# Autodesk Inventor assembly: ElectronicLoad
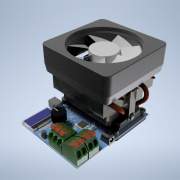
[picture p0: Inventor's stored thumbnail of the model, 180x180]
Saved by Autodesk Inventor 2021 (Build 250183000, 183)
## iProperties
Created: 2020-02-06
Part Number: ElectronicLoad
Document SubType Name: Assembly
Designer: Bradley
Author: Bradley
## Documents named in this file (42)
- C:\Users\Bradley\Documents\GitHub\Resources\Subsystems\Electronics\Testing\ElectronicLoad\CADModel\Native\ElectronicLoad.iam
- C:\Users\Bradley\Documents\GitHub\Resources\Subsystems\Electronics\Testing\ElectronicLoad\CADModel\Native\ElectronicLoad_PCB.ipt
- C:\Users\Bradley\Documents\GitHub\Resources\SupplierDocuments\05 - Connectors THT\05-0005\05-0005.ipt
- C:\Users\Bradley\Documents\GitHub\Resources\SupplierDocuments\05 - Connectors THT\05-0011\05-0011.ipt
- C:\Users\Bradley\Documents\GitHub\Resources\SupplierDocuments\05 - Connectors THT\05-0008\05-0008.ipt
- C:\Users\Bradley\Documents\GitHub\Resources\SupplierDocuments\05 - Connectors THT\05-0009\05-0009.ipt
- C:\Users\Bradley\Documents\GitHub\Resources\SupplierDocuments\04 - Connectors SMT\04-0004\04-0004.ipt
- C:\Users\Bradley\Documents\GitHub\Resources\SupplierDocuments\66 - Sensor\66-0006\66-0006.iam
- C:\Users\Bradley\Documents\GitHub\Resources\SupplierDocuments\03 - Board, Module, etc\03-0001\03-0001.ipt
- C:\Users\Bradley\Documents\GitHub\Resources\SupplierDocuments\05 - Connectors THT\05-0004\05-0004.ipt
- C:\Users\Bradley\Documents\GitHub\Resources\SupplierDocuments\61 - µController (and CLPD, FPGA,  etc.)\61-0002\61-0002.ipt
- C:\Users\Bradley\Documents\GitHub\Resources\SupplierDocuments\49 - Electromechanical\49-0005\49-0005.iam
- C:\Users\Bradley\Documents\GitHub\Resources\SupplierDocuments\48 - Hardware\48-0003\48-0003.iam
- C:\Users\Bradley\Documents\GitHub\Resources\SupplierDocuments\56 - Transistor FET\56-0008\56-0008-DOWN.ipt
- C:\Users\Bradley\Documents\GitHub\Resources\SupplierDocuments\23 - Resistor 3216\23-5m00\23-5m00.ipt
- C:\Users\Bradley\Documents\GitHub\Resources\SupplierDocuments\21 - Resistor 1608\21-0000\21-0000.ipt
- C:\Users\Bradley\Documents\GitHub\Resources\SupplierDocuments\36 - Ferrite\36-152A\36-152A.ipt
- C:\Users\Bradley\Documents\GitHub\Resources\SupplierDocuments\11 - Capacitor Ceramic 1608\11-105B\11-105B.ipt
- C:\Users\Bradley\Documents\GitHub\Resources\SupplierDocuments\21 - Resistor 1608\21-1001\21-1001.ipt
- C:\Users\Bradley\Documents\GitHub\Resources\SupplierDocuments\11 - Capacitor Ceramic 1608\11-102B\11-102B.ipt
- C:\Users\Bradley\Documents\GitHub\Resources\SupplierDocuments\16 - Capacitor Tantalum SMT\16-475A\16-475A.ipt
- C:\Users\Bradley\Documents\GitHub\Resources\SupplierDocuments\40 - Crystal SMT\40-805A\40-805A.ipt
- C:\Users\Bradley\Documents\GitHub\Resources\SupplierDocuments\21 - Resistor 1608\21-1002\21-1002.ipt
- C:\Users\Bradley\Documents\GitHub\Resources\SupplierDocuments\26 - Resistor Misc\26-0000\26-0000.ipt
- C:\Users\Bradley\Documents\GitHub\Resources\SupplierDocuments\11 - Capacitor Ceramic 1608\11-103A\11-103A.ipt
- C:\Users\Bradley\Documents\GitHub\Resources\SupplierDocuments\11 - Capacitor Ceramic 1608\11-100A\11-100A.ipt
- C:\Users\Bradley\Documents\GitHub\Resources\SupplierDocuments\21 - Resistor 1608\21-27.0\21-27.0.ipt
- C:\Users\Bradley\Documents\GitHub\Resources\SupplierDocuments\21 - Resistor 1608\21-3002\21-3002.ipt
- C:\Users\Bradley\Documents\GitHub\Resources\SupplierDocuments\21 - Resistor 1608\21-4702\21-4702.ipt
- C:\Users\Bradley\Documents\GitHub\Resources\SupplierDocuments\11 - Capacitor Ceramic 1608\11-470A\11-470A.ipt
- C:\Users\Bradley\Documents\GitHub\Resources\SupplierDocuments\21 - Resistor 1608\21-0.05\21-0.05.ipt
- C:\Users\Bradley\Documents\GitHub\Resources\SupplierDocuments\11 - Capacitor Ceramic 1608\11-104A\11-104A.ipt
- C:\Users\Bradley\Documents\GitHub\Resources\SupplierDocuments\21 - Resistor 1608\21-0.51\21-0.51.ipt
- C:\Users\Bradley\Documents\GitHub\Resources\SupplierDocuments\08 - Amplifier (excluding RF)\08-0002\08-0002.ipt
- C:\Users\Bradley\Documents\GitHub\Resources\SupplierDocuments\09 - Communication IC\09-0002\09-0002.ipt
- C:\Users\Bradley\Documents\GitHub\Resources\SupplierDocuments\63 - LED SMT\63-0001\63-0001.ipt
- C:\Users\Bradley\Documents\GitHub\Resources\SupplierDocuments\08 - Amplifier (excluding RF)\08-0003\08-0003.ipt
- C:\Users\Bradley\Documents\GitHub\Resources\SupplierDocuments\60 - Power IC\60-0009\60-0009.ipt
- C:\Users\Bradley\Documents\GitHub\Resources\SupplierDocuments\53 - Diode Misc\53-0001\53-0001.ipt
- C:\Users\Bradley\Documents\GitHub\Resources\SupplierDocuments\63 - LED SMT\63-0002\63-0002.ipt
- C:\Users\Bradley\Documents\GitHub\Resources\SupplierDocuments\56 - Transistor FET\56-0009\56-0009.ipt
- C:\Users\Bradley\Documents\GitHub\Resources\SupplierDocuments\60 - Power IC\60-0012\60-0012.ipt
## Components (90 placed, 41 different names)
1. ElectronicLoad_PCB:1 — Mate:6, Mate:7, Mate:8, Mate:9, Mate:10, Mate:11, Mate:12, Mate:13, Mate:14, Mate:15, Mate:16, Insert:1, Insert:2, Insert:3, Insert:4, Insert:5, Mate:27, Mate:34, Mate:35, Mate:36, Mate:37, Mate:38, Mate:39, Mate:50, Mate:53, Mate:55, Mate:56, Mate:57, Mate:58, Mate:59, Mate:60, Mate:61, Mate:62, Mate:63, Mate:64, Mate:75, Mate:76, Mate:77, Mate:78, Mate:79, Mate:80, Mate:81, Mate:95, Mate:96, Mate:99, Mate:100, Mate:105, Mate:106, Mate:108, Mate:109, Mate:110, Mate:111, Mate:120, Mate:121, Mate:125, Mate:127, Mate:128, Mate:133, Mate:134, Mate:139, Mate:140, Mate:141, Mate:148, Mate:150, Mate:151, Mate:156, Mate:158, Mate:159, Mate:160, Mate:161, Mate:162, Mate:163, Mate:164, Mate:165, Mate:166, Mate:167, Mate:168, Mate:169, Mate:186, Mate:189, Mate:191, Mate:194, Mate:195, Mate:200, Mate:201, Mate:204, Mate:207, Mate:208, Mate:209, Mate:212, Mate:213, Mate:215
2. 08-0002:1 — Mate:189, Mate:190, Flush:52
3. 09-0002:1 — Mate:191, Mate:192, Mate:193
4. 63-0001:1 — Mate:194, Mate:196, Mate:197
5. 63-0001:2 — Mate:195, Mate:198, Mate:199
6. 08-0003:1 — Mate:200, Mate:202, Mate:203
7. 08-0003:2 — Mate:201, Flush:53, Flush:54
8. 60-0009:1 — Mate:204, Mate:205, Mate:206
9. 53-0001:1 — Mate:207, Flush:55, Flush:56
10. 53-0001:2 — Mate:208, Flush:57, Flush:58
11. 63-0002:1 — Mate:209, Mate:210, Mate:211
12. 56-0009:1 — Mate:212, Mate:214, Flush:59
13. 56-0009:2 — Mate:213, Flush:60, Flush:61
14. 60-0012:1 — Mate:215, Flush:62, Flush:63
15. 21-0.51:1 — Mate:186, Mate:187, Mate:188
16. 11-104A:1 — Mate:158, Mate:170, Flush:44
17. 11-104A:2 — Mate:159, Mate:171, Mate:172
18. 11-104A:3 — Mate:160, Mate:173, Mate:174
19. 11-104A:4 — Mate:161, Mate:175, Mate:176
20. 11-104A:5 — Mate:162, Mate:177, Mate:178
21. 11-104A:6 — Mate:163, Mate:179, Flush:45
22. 11-104A:7 — Mate:164, Mate:180, Flush:46
23. 11-104A:8 — Mate:165, Mate:181, Flush:47
24. 11-104A:9 — Mate:166, Mate:182, Flush:48
25. 11-104A:10 — Mate:167, Mate:183, Flush:49
26. 11-104A:11 — Mate:168, Mate:184, Flush:50
27. 11-104A:12 — Mate:169, Mate:185, Flush:51
28. 21-0.05:1 — Mate:156, Mate:157, Flush:43
29. 11-470A:1 — Mate:150, Mate:152, Mate:153
30. 11-470A:2 — Mate:151, Mate:154, Mate:155
31. 21-4702:1 — Mate:148, Mate:149, Flush:42
32. 21-3002:1 — Mate:139, Mate:142, Mate:143
33. 21-3002:2 — Mate:140, Mate:144, Mate:145
34. 21-3002:3 — Mate:141, Mate:146, Mate:147
35. 21-27.0:1 — Mate:133, Mate:135, Mate:136
36. 21-27.0:2 — Mate:134, Mate:137, Mate:138
37. 11-100A:1 — Mate:127, Mate:129, Mate:130
38. 11-100A:2 — Mate:128, Mate:131, Mate:132
39. 11-103A:1 — Mate:125, Mate:126, Flush:41
40. 26-0000:1 — Mate:120, Mate:122, Flush:40
41. 26-0000:2 — Mate:121, Mate:123, Mate:124
42. 21-1002:1 — Mate:108, Mate:112, Mate:113
43. 21-1002:2 — Mate:109, Mate:114, Mate:115
44. 21-1002:3 — Mate:110, Mate:116, Mate:117
45. 21-1002:4 — Mate:111, Mate:118, Mate:119
46. 40-805A:1 — Mate:106, Mate:107, Flush:39
47. 23-5m00:2 — Mate:105, Flush:37, Flush:38
48. 16-475A:1 — Mate:99, Mate:101, Mate:102
49. 16-475A:2 — Mate:100, Mate:103, Mate:104
50. 11-102B:1 — Mate:95, Mate:97, Flush:35
51. 11-102B:2 — Mate:96, Mate:98, Flush:36
52. 21-1001:1 — Mate:75, Mate:82, Mate:83
53. 21-1001:2 — Mate:76, Mate:84, Mate:85
54. 21-1001:3 — Mate:77, Mate:86, Mate:87
55. 21-1001:4 — Mate:78, Mate:88, Mate:89
56. 21-1001:5 — Mate:79, Mate:90, Mate:91
57. 21-1001:6 — Mate:80, Mate:92, Mate:93
58. 21-1001:7 — Mate:81, Mate:94, Flush:34
59. 11-105B:1 — Mate:55, Mate:65, Flush:24
60. 11-105B:2 — Mate:56, Mate:66, Flush:25
61. 11-105B:3 — Mate:57, Mate:67, Flush:26
62. 11-105B:4 — Mate:58, Mate:68, Flush:27
63. 11-105B:5 — Mate:59, Mate:69, Flush:28
64. 11-105B:6 — Mate:60, Mate:70, Flush:29
65. 11-105B:7 — Mate:61, Mate:71, Flush:30
66. 11-105B:8 — Mate:62, Mate:72, Flush:31
67. 11-105B:9 — Mate:63, Mate:73, Flush:32
68. 11-105B:10 — Mate:64, Mate:74, Flush:33
69. 36-152A:1 — Mate:50, Mate:52, Flush:22
70. 36-152A:2 — Mate:53, Mate:54, Flush:23
71. 21-0000:1 — Mate:35, Mate:40, Flush:20
72. 21-0000:2 — Mate:36, Mate:41, Mate:42
73. 21-0000:3 — Mate:37, Mate:43, Mate:44
74. 21-0000:4 — Mate:38, Mate:45, Flush:21
75. 21-0000:5 — Mate:39, Mate:46, Mate:47
76. 23-5m00:1 — Mate:34, Flush:18, Flush:19
77. 05-0008:1 — Mate:8, Mate:30, Flush:16
78. 05-0008:2 — Mate:9, Mate:31, Flush:17
79. 05-0009:1 — Mate:6, Mate:32, Mate:33
80. 03-0001:1 — Mate:7, Flush:13, Flush:14
81. 66-0006:1 [sub-assembly] — Mate:11, Mate:23, Mate:24
82. 05-0005:1 — Mate:13, Mate:28, Mate:29
83. 05-0011:1 — Mate:12, Mate:26, Mate:27
84. 04-0004:1 — Mate:14, Flush:15, Mate:25
85. 05-0004:1 — Mate:10, Mate:22, Flush:12
86. 61-0002:1 — Mate:15, Mate:20, Mate:21
87. 49-0005:1 [sub-assembly] — Mate:16, Mate:18, Mate:19
88. 56-0008-DOWN:1 — Insert:4
89. 56-0008-DOWN:2 — Insert:5
90. 48-0003:1 [sub-assembly] — Insert:1, Insert:2, Insert:3
## Relationships (263: Mate 206, Flush 52, Insert 5)
- Mate:6: ElectronicLoad_PCB:1 ↔ 05-0009:1
- Mate:7: ElectronicLoad_PCB:1 ↔ 03-0001:1
- Mate:8: ElectronicLoad_PCB:1 ↔ 05-0008:1
- Mate:9: ElectronicLoad_PCB:1 ↔ 05-0008:2
- Mate:10: ElectronicLoad_PCB:1 ↔ 05-0004:1
- Mate:11 (1 mm): ElectronicLoad_PCB:1 ↔ 66-0006:1
- Mate:12: ElectronicLoad_PCB:1 ↔ 05-0011:1
- Mate:13: ElectronicLoad_PCB:1 ↔ 05-0005:1
- Mate:14: ElectronicLoad_PCB:1 ↔ 04-0004:1
- Mate:15: ElectronicLoad_PCB:1 ↔ 61-0002:1
- Mate:16: ElectronicLoad_PCB:1 ↔ 49-0005:1
- Insert:1: ElectronicLoad_PCB:1 ↔ 48-0003:1
- Insert:2: ElectronicLoad_PCB:1 ↔ 48-0003:1
- Insert:3: ElectronicLoad_PCB:1 ↔ 48-0003:1
- Insert:4: ElectronicLoad_PCB:1 ↔ 56-0008-DOWN:1
- Insert:5: ElectronicLoad_PCB:1 ↔ 56-0008-DOWN:2
- Mate:18 (-11 mm): 49-0005:1
- Mate:19 (-60.25 mm): 49-0005:1
- Mate:20 (4.75 mm): 61-0002:1
- Mate:21 (-11.45 mm): 61-0002:1
- Mate:22 (-44.5 mm): 05-0004:1
- Flush:12 (12.53 mm): 05-0004:1
- Flush:13 (43.75 mm): 03-0001:1
- Flush:14 (27.75 mm): 03-0001:1
- Mate:23 (-35 mm): 66-0006:1
- Mate:24 (-12 mm): 66-0006:1
- Flush:15 (37.85 mm): 04-0004:1
- Mate:25 (-37.45 mm): 04-0004:1
- Mate:26 (19.85 mm): 05-0011:1
- Mate:27: ElectronicLoad_PCB:1 ↔ 05-0011:1
- Mate:28 (-11.2 mm): 05-0005:1
- Mate:29 (43.5 mm): 05-0005:1
- Mate:30 (-42.5 mm): 05-0008:1
- Flush:16 (-47.5 mm): 05-0008:1
- Mate:31 (-60 mm): 05-0008:2
- Flush:17 (-47.35 mm): 05-0008:2
- Mate:32 (6.35 mm): 05-0009:1
- Mate:33 (-60 mm): 05-0009:1
- Mate:34: ElectronicLoad_PCB:1 ↔ 23-5m00:1
- Flush:18 (59.4 mm): 23-5m00:1
- Flush:19 (-40.95 mm): 23-5m00:1
- Mate:35: ElectronicLoad_PCB:1 ↔ 21-0000:1
- Mate:36: ElectronicLoad_PCB:1 ↔ 21-0000:2
- Mate:37: ElectronicLoad_PCB:1 ↔ 21-0000:3
- Mate:38: ElectronicLoad_PCB:1 ↔ 21-0000:4
- Mate:39: ElectronicLoad_PCB:1 ↔ 21-0000:5
- Mate:40 (-31.85 mm): 21-0000:1
- Flush:20 (-0.6 mm): 21-0000:1
- Mate:41 (-23.35 mm): 21-0000:2
- Mate:42 (-14.25 mm): 21-0000:2
- Mate:43 (-32.2 mm): 21-0000:3
- Mate:44 (-21 mm): 21-0000:3
- Mate:45 (-60.4 mm): 21-0000:4
- Flush:21 (25.55 mm): 21-0000:4
- Mate:46 (-35.1 mm): 21-0000:5
- Mate:47 (-21 mm): 21-0000:5
- Mate:50: ElectronicLoad_PCB:1 ↔ 36-152A:1
- Mate:52 (-35.85 mm): 36-152A:1
- Flush:22 (16.6 mm): 36-152A:1
- Mate:53: ElectronicLoad_PCB:1 ↔ 36-152A:2
- Mate:54 (-5.1 mm): 36-152A:2
- Flush:23 (21.4 mm): 36-152A:2
- Mate:55: ElectronicLoad_PCB:1 ↔ 11-105B:1
- Mate:56: ElectronicLoad_PCB:1 ↔ 11-105B:2
- Mate:57: ElectronicLoad_PCB:1 ↔ 11-105B:3
- Mate:58: ElectronicLoad_PCB:1 ↔ 11-105B:4
- Mate:59: ElectronicLoad_PCB:1 ↔ 11-105B:5
- Mate:60: ElectronicLoad_PCB:1 ↔ 11-105B:6
- Mate:61: ElectronicLoad_PCB:1 ↔ 11-105B:7
- Mate:62: ElectronicLoad_PCB:1 ↔ 11-105B:8
- Mate:63: ElectronicLoad_PCB:1 ↔ 11-105B:9
- Mate:64: ElectronicLoad_PCB:1 ↔ 11-105B:10
- Mate:65 (-25 mm): 11-105B:1
- Flush:24 (50.55 mm): 11-105B:1
- Mate:66 (-25 mm): 11-105B:2
- Flush:25 (52.25 mm): 11-105B:2
- Mate:67 (-25 mm): 11-105B:3
- Flush:26 (53.95 mm): 11-105B:3
- Mate:68 (-25 mm): 11-105B:4
- Flush:27 (55.65 mm): 11-105B:4
- Mate:69 (-24.95 mm): 11-105B:5
- Flush:28 (42.5 mm): 11-105B:5
- Mate:70 (-25 mm): 11-105B:6
- Flush:29 (48.75 mm): 11-105B:6
- Mate:71 (17.05 mm): 11-105B:7
- Flush:30 (28.55 mm): 11-105B:7
- Mate:72 (13.05 mm): 11-105B:8
- Flush:31 (20.8 mm): 11-105B:8
- Mate:73 (-27.85 mm): 11-105B:9
- Flush:32 (5.45 mm): 11-105B:9
- Mate:74 (-34.25 mm): 11-105B:10
- Flush:33 (7.45 mm): 11-105B:10
- Mate:75: ElectronicLoad_PCB:1 ↔ 21-1001:1
- Mate:76: ElectronicLoad_PCB:1 ↔ 21-1001:2
- Mate:77: ElectronicLoad_PCB:1 ↔ 21-1001:3
- Mate:78: ElectronicLoad_PCB:1 ↔ 21-1001:4
- Mate:79: ElectronicLoad_PCB:1 ↔ 21-1001:5
- Mate:80: ElectronicLoad_PCB:1 ↔ 21-1001:6
- Mate:81: ElectronicLoad_PCB:1 ↔ 21-1001:7
- Mate:82 (-14.05 mm): 21-1001:1
- Mate:83 (-14.7 mm): 21-1001:1
- Mate:84 (-15.15 mm): 21-1001:2
- Mate:85 (-5.25 mm): 21-1001:2
- Mate:86 (-19.5 mm): 21-1001:3
- Mate:87 (-11.5 mm): 21-1001:3
- Mate:88 (-3.55 mm): 21-1001:4
- Mate:89 (-24.65 mm): 21-1001:4
- Mate:90 (27.85 mm): 21-1001:5
- Mate:91 (-29.3 mm): 21-1001:5
- Mate:92 (-3.9 mm): 21-1001:6
- Mate:93 (-56 mm): 21-1001:6
- Mate:94 (-35.8 mm): 21-1001:7
- Flush:34 (-4.2 mm): 21-1001:7
- Mate:95: ElectronicLoad_PCB:1 ↔ 11-102B:1
- Mate:96: ElectronicLoad_PCB:1 ↔ 11-102B:2
- Mate:97 (-25 mm): 11-102B:1
- Flush:35 (46.95 mm): 11-102B:1
- Mate:98 (-24.95 mm): 11-102B:2
- Flush:36 (44.2 mm): 11-102B:2
- Mate:99: ElectronicLoad_PCB:1 ↔ 16-475A:1
- Mate:100: ElectronicLoad_PCB:1 ↔ 16-475A:2
- Mate:101 (-10.95 mm): 16-475A:1
- Mate:102 (-21.6 mm): 16-475A:1
- Mate:103 (-28.1 mm): 16-475A:2
- Mate:104 (-17.15 mm): 16-475A:2
- Mate:105: ElectronicLoad_PCB:1 ↔ 23-5m00:2
- Flush:37 (-34.8 mm): 23-5m00:2
- Flush:38 (28.4 mm): 23-5m00:2
- Mate:106: ElectronicLoad_PCB:1 ↔ 40-805A:1
- Mate:107 (2.55 mm): 40-805A:1
- Flush:39 (21.05 mm): 40-805A:1
- Mate:108: ElectronicLoad_PCB:1 ↔ 21-1002:1
- Mate:109: ElectronicLoad_PCB:1 ↔ 21-1002:2
- Mate:110: ElectronicLoad_PCB:1 ↔ 21-1002:3
- Mate:111: ElectronicLoad_PCB:1 ↔ 21-1002:4
- Mate:112 (-3.9 mm): 21-1002:1
- Mate:113 (-50.9 mm): 21-1002:1
- Mate:114 (-3.9 mm): 21-1002:2
- Mate:115 (-52.6 mm): 21-1002:2
- Mate:116 (-20 mm): 21-1002:3
- Mate:117 (-15.4 mm): 21-1002:3
- Mate:118 (-31.05 mm): 21-1002:4
- Mate:119 (3 mm): 21-1002:4
- Mate:120: ElectronicLoad_PCB:1 ↔ 26-0000:1
- Mate:121: ElectronicLoad_PCB:1 ↔ 26-0000:2
- Mate:122 (-12.55 mm): 26-0000:1
- Flush:40 (8.95 mm): 26-0000:1
- Mate:123 (-18.6 mm): 26-0000:2
- Mate:124 (-59.95 mm): 26-0000:2
- Mate:125: ElectronicLoad_PCB:1 ↔ 11-103A:1
- Mate:126 (-23.35 mm): 11-103A:1
- Flush:41 (16.15 mm): 11-103A:1
- Mate:127: ElectronicLoad_PCB:1 ↔ 11-100A:1
- Mate:128: ElectronicLoad_PCB:1 ↔ 11-100A:2
- Mate:129 (-24.85 mm): 11-100A:1
- Mate:130 (5.5 mm): 11-100A:1
- Mate:131 (-24.9 mm): 11-100A:2
- Mate:132 (3.75 mm): 11-100A:2
- Mate:133: ElectronicLoad_PCB:1 ↔ 21-27.0:1
- Mate:134: ElectronicLoad_PCB:1 ↔ 21-27.0:2
- Mate:135 (-34.15 mm): 21-27.0:1
- Mate:136 (-11.1 mm): 21-27.0:1
- Mate:137 (-34.15 mm): 21-27.0:2
- Mate:138 (-13.5 mm): 21-27.0:2
- Mate:139: ElectronicLoad_PCB:1 ↔ 21-3002:1
- Mate:140: ElectronicLoad_PCB:1 ↔ 21-3002:2
- Mate:141: ElectronicLoad_PCB:1 ↔ 21-3002:3
- Mate:142 (-3.9 mm): 21-3002:1
- Mate:143 (-49.2 mm): 21-3002:1
- Mate:144 (-3.9 mm): 21-3002:2
- Mate:145 (-54.3 mm): 21-3002:2
- Mate:146 (-33.1 mm): 21-3002:3
- Mate:147 (-5.7 mm): 21-3002:3
- Mate:148: ElectronicLoad_PCB:1 ↔ 21-4702:1
- Mate:149 (-32.35 mm): 21-4702:1
- Flush:42 (-7.3 mm): 21-4702:1
- Mate:150: ElectronicLoad_PCB:1 ↔ 11-470A:1
- Mate:151: ElectronicLoad_PCB:1 ↔ 11-470A:2
- Mate:152 (-12.9 mm): 11-470A:1
- Mate:153 (-36.45 mm): 11-470A:1
- Mate:154 (-10 mm): 11-470A:2
- Mate:155 (-36.45 mm): 11-470A:2
- Mate:156: ElectronicLoad_PCB:1 ↔ 21-0.05:1
- Mate:157 (-26.6 mm): 21-0.05:1
- Flush:43 (-30.05 mm): 21-0.05:1
- Mate:158: ElectronicLoad_PCB:1 ↔ 11-104A:1
- Mate:159: ElectronicLoad_PCB:1 ↔ 11-104A:2
- Mate:160: ElectronicLoad_PCB:1 ↔ 11-104A:3
- Mate:161: ElectronicLoad_PCB:1 ↔ 11-104A:4
- Mate:162: ElectronicLoad_PCB:1 ↔ 11-104A:5
- Mate:163: ElectronicLoad_PCB:1 ↔ 11-104A:6
- Mate:164: ElectronicLoad_PCB:1 ↔ 11-104A:7
- Mate:165: ElectronicLoad_PCB:1 ↔ 11-104A:8
- Mate:166: ElectronicLoad_PCB:1 ↔ 11-104A:9
- Mate:167: ElectronicLoad_PCB:1 ↔ 11-104A:10
- Mate:168: ElectronicLoad_PCB:1 ↔ 11-104A:11
- Mate:169: ElectronicLoad_PCB:1 ↔ 11-104A:12
- Mate:170 (-0.15 mm): 11-104A:1
- Flush:44 (3.85 mm): 11-104A:1
- Mate:171 (-8.35 mm): 11-104A:2
- Mate:172 (12.35 mm): 11-104A:2
- Mate:173 (-15.15 mm): 11-104A:3
- Mate:174 (12.35 mm): 11-104A:3
- Mate:175 (-27.45 mm): 11-104A:4
- Mate:176 (-0.15 mm): 11-104A:4
- Mate:177 (-16.3 mm): 11-104A:5
- Mate:178 (-2.85 mm): 11-104A:5
- Mate:179 (12 mm): 11-104A:6
- Flush:45 (33.05 mm): 11-104A:6
- Mate:180 (19 mm): 11-104A:7
- Flush:46 (15.65 mm): 11-104A:7
- Mate:181 (17.8 mm): 11-104A:8
- Flush:47 (24.75 mm): 11-104A:8
- Mate:182 (-24.95 mm): 11-104A:9
- Flush:48 (40.75 mm): 11-104A:9
- Mate:183 (-11.25 mm): 11-104A:10
- Flush:49 (5.25 mm): 11-104A:10
- Mate:184 (-22.7 mm): 11-104A:11
- Flush:50 (19.25 mm): 11-104A:11
- Mate:185 (-34.15 mm): 11-104A:12
- Flush:51 (9.4 mm): 11-104A:12
- Mate:186: ElectronicLoad_PCB:1 ↔ 21-0.51:1
- Mate:187 (27.7 mm): 21-0.51:1
- Mate:188 (-26 mm): 21-0.51:1
- Mate:189: ElectronicLoad_PCB:1 ↔ 08-0002:1
- Mate:190 (23 mm): 08-0002:1
- Flush:52 (34.9 mm): 08-0002:1
- Mate:191: ElectronicLoad_PCB:1 ↔ 09-0002:1
- Mate:192 (-11.9 mm): 09-0002:1
- Mate:193 (-30.1 mm): 09-0002:1
- Mate:194: ElectronicLoad_PCB:1 ↔ 63-0001:1
- Mate:195: ElectronicLoad_PCB:1 ↔ 63-0001:2
- Mate:196 (3.05 mm): 63-0001:1
- Mate:197 (-29.65 mm): 63-0001:1
- Mate:198 (-16.5 mm): 63-0001:2
- Mate:199 (-11.5 mm): 63-0001:2
- Mate:200: ElectronicLoad_PCB:1 ↔ 08-0003:1
- Mate:201: ElectronicLoad_PCB:1 ↔ 08-0003:2
- Mate:202 (-20.5 mm): 08-0003:1
- Mate:203 (17.85 mm): 08-0003:1
- Flush:53 (17.4 mm): 08-0003:2
- Flush:54 (-22.3 mm): 08-0003:2
- Mate:204: ElectronicLoad_PCB:1 ↔ 60-0009:1
- Mate:205 (-25.15 mm): 60-0009:1
- Mate:206 (13.65 mm): 60-0009:1
- Mate:207: ElectronicLoad_PCB:1 ↔ 53-0001:1
- Mate:208: ElectronicLoad_PCB:1 ↔ 53-0001:2
- Flush:55 (1 mm): 53-0001:1
- Flush:56 (27.15 mm): 53-0001:1
- Flush:57 (-3.1 mm): 53-0001:2
- Flush:58 (27.25 mm): 53-0001:2
- Mate:209: ElectronicLoad_PCB:1 ↔ 63-0002:1
- Mate:210 (-16.5 mm): 63-0002:1
- Mate:211 (-9.7 mm): 63-0002:1
- Mate:212: ElectronicLoad_PCB:1 ↔ 56-0009:1
- Mate:213: ElectronicLoad_PCB:1 ↔ 56-0009:2
- Mate:214 (26.85 mm): 56-0009:1
- Flush:59 (22 mm): 56-0009:1
- Flush:60 (22.55 mm): 56-0009:2
- Flush:61 (-34 mm): 56-0009:2
- Mate:215: ElectronicLoad_PCB:1 ↔ 60-0012:1
- Flush:62 (0.7 mm): 60-0012:1
- Flush:63 (32.45 mm): 60-0012:1
